# Autodesk Inventor assembly: part assemble
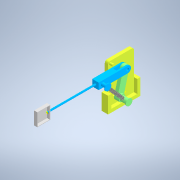
[picture p0: Inventor's stored thumbnail of the model, 180x180]
Saved by Autodesk Inventor 2021 (Build 250183000, 183)
## iProperties
Created: 2021-07-09
Part Number: part assemble
Document SubType Name: Assembly
Designer: HP
Author: HP
## Documents named in this file (6)
- D:\exploration\part assemble.iam
- C:\Users\HP\Documents\Part1....ipt
- C:\Users\HP\Documents\Part2.ipt
- C:\Users\HP\Documents\Part3.ipt
- C:\Users\HP\Documents\Part4.ipt
- C:\Users\HP\Documents\part6.ipt
## Components (5 placed, 5 different names)
1. Part1...:1 — Mate:1, Mate:2
2. Part2:1 — Mate:3, Mate:4, Mate:6
3. Part3:1 — Mate:1, Mate:2, Mate:3, Mate:4, Mate:5, Mate:7
4. Part4:1 — Mate:5
5. part6:1 — Mate:6, Mate:7
## Relationships (7: Mate 7)
- Mate:1: Part1...:1 ↔ Part3:1
- Mate:2: Part1...:1 ↔ Part3:1
- Mate:3: Part2:1 ↔ Part3:1
- Mate:4: Part2:1 ↔ Part3:1
- Mate:5: Part3:1 ↔ Part4:1
- Mate:6: Part2:1 ↔ part6:1
- Mate:7: Part3:1 ↔ part6:1
